# Autodesk Inventor assembly: 오른허벅지
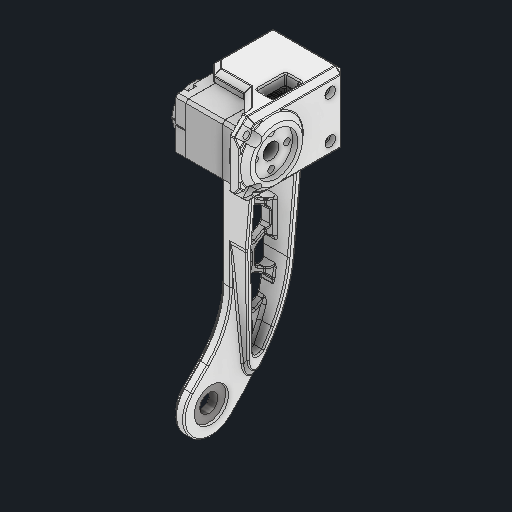
[picture p0: Inventor's stored thumbnail of the model, 512x512]
Saved by Autodesk Inventor 2027.1 (Build 311270010, 270A)
## iProperties
Created: 2026-08-22
Part Number: 오른허벅지
Document SubType Name: Assembly
Designer: moieboy9999
Mass: 46 g
Surface Area: 420.118 cm^2
Volume: 61.3166 cm^3
Density: 0.750205 g/cm^3
Author: moieboy9999
## Documents named in this file (4)
- D:\micro_dog_cad\다리\프레임\오른허벅지.iam
- D:\micro_dog_cad\다리\프레임\허벅지_MIR.ipt
- D:\micro_dog_cad\부품\XL,XC-330.ipt
- D:\micro_dog_cad\부품\큰베어링.ipt
## Components (3 placed, 3 different names)
1. 허벅지_MIR:1 — 메이트:1, 플러쉬:1, 메이트:2, 메이트:3
2. XL,XC-330:1 — 메이트:2, 메이트:3
3. 큰베어링:1 — 메이트:1, 플러쉬:1
## Relationships (4: Mate 3, Flush 1)
- 메이트:1 [Mate]: 허벅지_MIR:1 ↔ 큰베어링:1
- 플러쉬:1 [Flush] (1 mm): 허벅지_MIR:1 ↔ 큰베어링:1
- 메이트:2 [Mate]: 허벅지_MIR:1 ↔ XL,XC-330:1
- 메이트:3 [Mate]: 허벅지_MIR:1 ↔ XL,XC-330:1
